# Autodesk Inventor assembly: printer
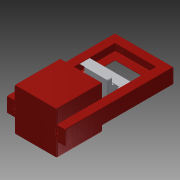
[picture p0: Inventor's stored thumbnail of the model, 180x180]
Saved by Autodesk Inventor 2014 SP2 (Build 180246200, 246)
## iProperties
Created: 2016-09-18
Part Number: printer
Document SubType Name: Assembly
Designer: cruiser
Mass: 7025.38 g
Surface Area: 12453 cm^2
Volume: 1064.35 cm^3
Density: 6.60061 g/cm^3
Author: cruiser
## Documents named in this file (8)
- C:\Users\cruiser\Desktop\models\3d printers\laserresin5\printer.iam
- C:\Users\cruiser\Desktop\models\3d printers\laserresin5\frame_front.ipt
- C:\Users\cruiser\Desktop\models\3d printers\laserresin5\frame_back.ipt
- C:\Users\cruiser\Desktop\models\3d printers\laserresin5\drawer.ipt
- C:\Users\cruiser\Desktop\models\3d printers\laserresin5\reservoir.ipt
- C:\Users\cruiser\Desktop\models\3d printers\laserresin5\tray.ipt
- C:\Users\cruiser\Desktop\models\3d printers\laserresin5\crane.ipt
- C:\Users\cruiser\Desktop\models\3d printers\laserresin5\platform.ipt
## Components (8 placed, 7 different names)
1. frame_front:1 — Flush:1, Flush:2, Mate:1, Mate:2, Mate:8, Mate:9, Mate:10
2. frame_back:1 — Flush:1, Flush:2, Mate:11
3. drawer:1 — Mate:1, Mate:7, Mate:10
4. drawer:2 — Mate:2, Mate:11
5. reservoir:1 — Mate:5, Flush:3, Flush:4, Mate:7
6. tray:1 — Mate:5, Flush:3, Flush:4
7. crane:1 — Mate:6, Flush:5, Mate:8, Mate:9
8. platform:1 — Mate:6, Flush:5
## Relationships (14: Mate 9, Flush 5)
- Flush:1: frame_front:1 ↔ frame_back:1
- Flush:2: frame_front:1 ↔ frame_back:1
- Mate:1: frame_front:1 ↔ drawer:1
- Mate:2: frame_front:1 ↔ drawer:2
- Mate:5: reservoir:1 ↔ tray:1
- Flush:3: reservoir:1 ↔ tray:1
- Flush:4: reservoir:1 ↔ tray:1
- Mate:6: crane:1 ↔ platform:1
- Flush:5: crane:1 ↔ platform:1
- Mate:7: drawer:1 ↔ reservoir:1
- Mate:8: frame_front:1 ↔ crane:1
- Mate:9: frame_front:1 ↔ crane:1
- Mate:10: frame_front:1 ↔ drawer:1
- Mate:11: frame_back:1 ↔ drawer:2
